# Autodesk Inventor assembly: Swerve Drive
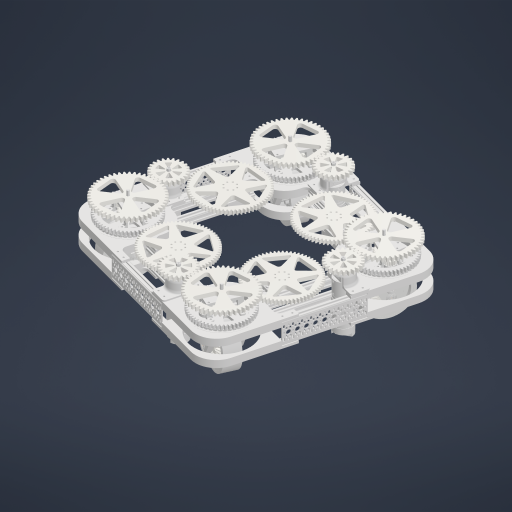
[picture p0: Inventor's stored thumbnail of the model, 512x512]
Saved by Autodesk Inventor 2023 (Build 270158000, 158)
## iProperties
Created: 2022-11-20
Part Number: Swerve Drive
Document SubType Name: Assembly
Designer: Izack Waczko
Author: Izack Waczko
## Documents named in this file (2)
- D:\Robotics\Custom-Modules-CAD\Custom-Swerve-Drive\Version 1\Swerve Drive V1.iam
- D:\Robotics\Custom-Modules-CAD\Custom-Swerve-Drive\Version 1\Swerve Module V1.iam
## Components (4 placed, 1 different names)
1. Swerve Module V1:1 [sub-assembly] — Flush:1, Mate:1, Mate:2, Flush:4
2. Swerve Module V1:2 [sub-assembly] — Flush:1, Mate:1, Mate:2, Mate:3, Mate:6, Flush:2
3. Swerve Module V1:3 [sub-assembly] — Mate:3, Mate:4, Mate:5, Mate:6, Flush:2, Flush:3
4. Swerve Module V1:4 [sub-assembly] — Mate:4, Mate:5, Flush:3, Flush:4
## Relationships (10: Mate 6, Flush 4)
- Flush:1: Swerve Module V1:1 ↔ Swerve Module V1:2
- Mate:1: Swerve Module V1:1 ↔ Swerve Module V1:2
- Mate:2: Swerve Module V1:1 ↔ Swerve Module V1:2
- Mate:3: Swerve Module V1:2 ↔ Swerve Module V1:3
- Mate:4: Swerve Module V1:3 ↔ Swerve Module V1:4
- Mate:5: Swerve Module V1:3 ↔ Swerve Module V1:4
- Mate:6: Swerve Module V1:2 ↔ Swerve Module V1:3
- Flush:2: Swerve Module V1:2 ↔ Swerve Module V1:3
- Flush:3: Swerve Module V1:3 ↔ Swerve Module V1:4
- Flush:4: Swerve Module V1:1 ↔ Swerve Module V1:4
